# Autodesk Inventor assembly: VersaPlanetary (Fixed)
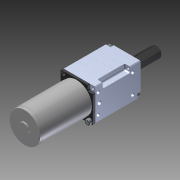
[picture p0: Inventor's stored thumbnail of the model, 180x180]
Saved by Autodesk Inventor 2014 (Build 180170000, 170)
## iProperties
Created: 2014-01-13
Part Number: VersaPlanetary (Fixed)
Document SubType Name: Assembly
Designer: motoennies
Title: 217-2 Stage Versaplanetary STEP.STEP
Description: STEP AP214
Creation Date: 2013-12-10
Sending System: SolidWorks 2013
Preprocessor: SwSTEP 2.0
Author: motoennies
## Documents named in this file (18)
- \\NNHSSRV2.hs.sd203.org\MOToennies$\Robotics\2014buildCAD-master\Collector\VersaPlanetary (Fixed).iam
- \\NNHSSRV2.hs.sd203.org\MOToennies$\Inventor\217-2625-001 Rev1.ipt
- \\NNHSSRV2.hs.sd203.org\MOToennies$\Inventor\217-2625-002 Rev1.ipt
- \\NNHSSRV2.hs.sd203.org\MOToennies$\Inventor\217-2625-003 Rev1.ipt
- \\NNHSSRV2.hs.sd203.org\MOToennies$\Inventor\217-2625-009 Rev1.ipt
- \\NNHSSRV2.hs.sd203.org\MOToennies$\Inventor\217-2816-001 Rev1.ipt
- \\NNHSSRV2.hs.sd203.org\MOToennies$\Inventor\217-2625-007 Rev1_Sun_Driver01.ipt
- \\NNHSSRV2.hs.sd203.org\MOToennies$\Inventor\217-2625-100.iam
- \\NNHSSRV2.hs.sd203.org\MOToennies$\Inventor\217-2822-003 Rev4.ipt
- \\NNHSSRV2.hs.sd203.org\MOToennies$\Inventor\217-2625-011 Rev1.ipt
- \\NNHSSRV2.hs.sd203.org\MOToennies$\Inventor\SSA_SSA0832-0500ZC.ipt
- \\NNHSSRV2.hs.sd203.org\MOToennies$\Inventor\217-2742.ipt
- \\NNHSSRV2.hs.sd203.org\MOToennies$\Inventor\SSA_SSA0832-1750ZC.ipt
- \\NNHSSRV2.hs.sd203.org\MOToennies$\Inventor\217-2625-018 Rev1_98541A410.ipt
- \\NNHSSRV2.hs.sd203.org\MOToennies$\Inventor\217-2625-017 Rev1_9714K61.ipt
- \\NNHSSRV2.hs.sd203.org\MOToennies$\Inventor\PINL-M020-006-S.ipt
- \\NNHSSRV2.hs.sd203.org\MOToennies$\Inventor\217-3106-000 Rev2_NO SUN.iam
- \\NNHSSRV2.hs.sd203.org\MOToennies$\Robotics\2014buildCAD-master\Collector\BAG Motor.ipt
## Components (21 placed, 21 different names)
1. 217-2625-001 Rev1_1
2. 217-2625-002 Rev1_2
3. 217-2625-003 Rev1_3
4. 217-2625-009 Rev1_4
5. 217-2816-001 Rev1_5
6. 217-2625-007 Rev1_Sun_Driver01_6
7. 217-2625-100_7 [sub-assembly]
8. 217-2822-003 Rev4_8 — Insert:1, Insert:2
9. 217-2625-011 Rev1_9
10. SSA_SSA0832-0500ZC_10
11. 217-2742_11
12. 217-2742_12
13. SSA_SSA0832-1750ZC_13
14. SSA_SSA0832-1750ZC_14
15. 217-2625-018 Rev1_98541A410_15
16. 217-2625-017 Rev1_9714K61_16
17. PINL-M020-006-S_17
18. PINL-M020-006-S_18
19. 217-2816-001 Rev1_20
20. 217-3106-000 Rev2_NO SUN_21 [sub-assembly]
21. BAG Motor:1 — Insert:1, Insert:2
## Relationships (2: Insert 2)
- Insert:1: 217-2822-003 Rev4_8 ↔ BAG Motor:1
- Insert:2: 217-2822-003 Rev4_8 ↔ BAG Motor:1
